# Autodesk Inventor assembly: bayonet connector
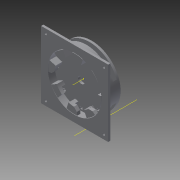
[picture p0: Inventor's stored thumbnail of the model, 180x180]
Saved by Autodesk Inventor 2015 (Build 190159000, 159)
## iProperties
Created: 2014-09-30
Part Number: bayonet connector
Document SubType Name: Assembly
Designer: ericd_000
Author: ericd_000
## Documents named in this file (4)
- C:\Users\ericd_000\Dropbox\GitHub\initial_cad\eric_cad\bayonet connector.iam
- C:\Users\ericd_000\Dropbox\GitHub\initial_cad\eric_cad\bayonet container 8.ipt
- C:\Users\ericd_000\Downloads\Imported Components\1561T270 (1)\1561T270 (1).ipt
- C:\Users\ericd_000\Dropbox\GitHub\initial_cad\eric_cad\inner bayonet connector 8mk2.ipt
## Components (3 placed, 3 different names)
1. bayonet container 8:1 — Mate:2, Mate:3
2. 1561T270 (1):1
3. inner bayonet connector 8mk2:1 — Mate:2, Mate:3
## Relationships (2: Mate 2)
- Mate:2: bayonet container 8:1 ↔ inner bayonet connector 8mk2:1
- Mate:3: bayonet container 8:1 ↔ inner bayonet connector 8mk2:1
